# Autodesk Inventor assembly: Anemometr
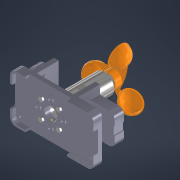
[picture p0: Inventor's stored thumbnail of the model, 180x180]
Saved by Autodesk Inventor 2021.2 (Build 252289000, 289)
## iProperties
Created: 2021-10-17
Part Number: Anemometr
Document SubType Name: Assembly
Designer: DuctopwH
Author: DuctopwH
## Documents named in this file (18)
- F:\Projects\cadblueprints\002-АНМ\002-ANM.iam
- F:\Projects\cadblueprints\002-АНМ\parts\002.10-plita.ipt
- F:\Projects\cadblueprints\002-АНМ\parts\002.09-flanec.ipt
- F:\Projects\cadblueprints\002-АНМ\parts\002.01-korpus.ipt
- F:\Projects\cadblueprints\002-АНМ\parts\002.02-osnovanie.ipt
- C:\Users\DuctopwH\Documents\Inventor\Content Center Files\R2021\en-US\Bolt GOST R 50274-92\Bolt M5-6g×16-F GOST R 50274-92.ipt
- F:\Projects\cadblueprints\002-АНМ\parts\002.04-terminal.ipt
- C:\Users\DuctopwH\Documents\Inventor\Content Center Files\R2021\en-US\GOST 10450-78\Washer 2,7 GOST 10450-78.ipt
- C:\Users\DuctopwH\Documents\Inventor\Content Center Files\R2021\en-US\GOST 5916-70\Nut M2,5-6H GOST 5916-70.ipt
- F:\Projects\cadblueprints\002-АНМ\parts\002.08-kryshka.ipt
- F:\Projects\cadblueprints\002-АНМ\standard-parts\ANSI B18.3.1M - M2,5x0,45 x 12.ipt
- F:\Projects\cadblueprints\002-АНМ\standard-parts\DIN 988 - S4 x 8.ipt
- F:\Projects\cadblueprints\002-АНМ\parts\002.06-rotor.ipt
- F:\Projects\cadblueprints\002-АНМ\parts\002.05-val.ipt
- F:\Projects\cadblueprints\002-АНМ\parts\002.03-vtulka.ipt
- F:\Projects\cadblueprints\002-АНМ\standard-parts\Ring 8 GOST 13943-86.ipt
- F:\Projects\cadblueprints\002-АНМ\parts\002.07-krylchatka.ipt
- C:\Users\DuctopwH\Documents\Inventor\Content Center Files\R2021\en-US\Bolt GOST R 50792-95\Bolt M5×20 GOST R 50792-95.ipt
## Components (26 placed, 17 different names)
1. 002.10-plita:1 — Mate:1, Flush:1, Flush:2, Mate:2, Mate:3, Mate:4, Mate:6, Mate:7, Insert:3, Insert:4, Insert:5, Insert:6
2. 002.09-flanec:1 — Mate:2, Mate:3, Mate:4, Mate:5
3. 002.01-korpus:1 — Mate:5, Mate:6, Mate:7, Mate:8, Mate:9, Mate:10, Insert:1, Insert:2, Mate:25, Mate:26, Mate:27, Mate:29, Mate:31
4. 002.02-osnovanie:1 — Mate:8, Mate:9, Mate:10, Mate:11, Mate:12, Mate:15, Mate:16, Mate:18, Mate:20, Mate:32, Mate:33, Mate:34, Mate:38, Mate:49, Mate:50
5. Bolt GOST R 50274-92 M5-6g×16-F:1 — Insert:1
6. Bolt GOST R 50274-92 M5-6g×16-F:2 — Insert:2
7. 002.04-terminal:1 — Mate:12, Mate:16, Mate:19, Mate:23, Mate:49
8. 002.04-terminal:2 — Mate:11, Mate:15, Mate:17, Mate:21, Mate:50
9. Washer GOST 10450-78 2,7:1 — Mate:17, Mate:18, Mate:22
10. Washer GOST 10450-78 2,7:2 — Mate:19, Mate:20, Mate:24
11. Nut GOST 5916-70 M2,5:1 — Mate:21, Mate:22
12. Nut GOST 5916-70 M2,5:2 — Mate:23, Mate:24
13. 002.08-kryshka:1 — Mate:25, Mate:26, Mate:27, Mate:28, Mate:30, Flush:3, Mate:42, Mate:43, Mate:46, Mate:48
14. Broached Socket Head Cap Screw - Metric M2,5x0,45 x 12:1 — Mate:28, Mate:29
15. Broached Socket Head Cap Screw - Metric M2,5x0,45 x 12:2 — Mate:30, Mate:31
16. DIN 988 S4 x 8:1 — Mate:32, Mate:33, Mate:36
17. 002.06-rotor:1 — Mate:34, Mate:35, Mate:36
18. 002.05-val:1 — Mate:38, Mate:39, Mate:40, Mate:44
19. 002.03-vtulka:1 — Mate:39, Flush:3, Mate:41
20. 002.03-vtulka:2 — Mate:40, Mate:41
21. Ring GOST 13943-86 A 8:1 — Mate:47, Mate:48
22. 002.07-krylchatka:1 — Mate:42, Mate:43, Mate:44, Mate:46, Mate:47
23. Bolt GOST R 50792-95 M5×20:1 — Insert:3
24. Bolt GOST R 50792-95 M5×20:2 — Insert:4
25. Bolt GOST R 50792-95 M5×20:3 — Insert:5
26. Bolt GOST R 50792-95 M5×20:4 — Insert:6
## Relationships (55: Mate 46, Insert 6, Flush 3)
- Mate:1: 002.10-plita:1
- Flush:1: 002.10-plita:1
- Flush:2: 002.10-plita:1
- Mate:2: 002.10-plita:1 ↔ 002.09-flanec:1
- Mate:3: 002.10-plita:1 ↔ 002.09-flanec:1
- Mate:4: 002.10-plita:1 ↔ 002.09-flanec:1
- Mate:5: 002.09-flanec:1 ↔ 002.01-korpus:1
- Mate:6: 002.10-plita:1 ↔ 002.01-korpus:1
- Mate:7: 002.10-plita:1 ↔ 002.01-korpus:1
- Mate:8: 002.01-korpus:1 ↔ 002.02-osnovanie:1
- Mate:9: 002.01-korpus:1 ↔ 002.02-osnovanie:1
- Mate:10: 002.01-korpus:1 ↔ 002.02-osnovanie:1
- Insert:1: 002.01-korpus:1 ↔ Bolt GOST R 50274-92 M5-6g×16-F:1
- Insert:2: 002.01-korpus:1 ↔ Bolt GOST R 50274-92 M5-6g×16-F:2
- Mate:11: 002.02-osnovanie:1 ↔ 002.04-terminal:2
- Mate:12: 002.02-osnovanie:1 ↔ 002.04-terminal:1
- Mate:15: 002.02-osnovanie:1 ↔ 002.04-terminal:2
- Mate:16: 002.02-osnovanie:1 ↔ 002.04-terminal:1
- Mate:17: 002.04-terminal:2 ↔ Washer GOST 10450-78 2,7:1
- Mate:18: 002.02-osnovanie:1 ↔ Washer GOST 10450-78 2,7:1
- Mate:19: 002.04-terminal:1 ↔ Washer GOST 10450-78 2,7:2
- Mate:20: 002.02-osnovanie:1 ↔ Washer GOST 10450-78 2,7:2
- Mate:21: 002.04-terminal:2 ↔ Nut GOST 5916-70 M2,5:1
- Mate:22: Washer GOST 10450-78 2,7:1 ↔ Nut GOST 5916-70 M2,5:1
- Mate:23: 002.04-terminal:1 ↔ Nut GOST 5916-70 M2,5:2
- Mate:24: Washer GOST 10450-78 2,7:2 ↔ Nut GOST 5916-70 M2,5:2
- Mate:25: 002.01-korpus:1 ↔ 002.08-kryshka:1
- Mate:26: 002.01-korpus:1 ↔ 002.08-kryshka:1
- Mate:27: 002.01-korpus:1 ↔ 002.08-kryshka:1
- Mate:28: 002.08-kryshka:1 ↔ Broached Socket Head Cap Screw - Metric M2,5x0,45 x 12:1
- Mate:29: 002.01-korpus:1 ↔ Broached Socket Head Cap Screw - Metric M2,5x0,45 x 12:1
- Mate:30: 002.08-kryshka:1 ↔ Broached Socket Head Cap Screw - Metric M2,5x0,45 x 12:2
- Mate:31: 002.01-korpus:1 ↔ Broached Socket Head Cap Screw - Metric M2,5x0,45 x 12:2
- Mate:32: 002.02-osnovanie:1 ↔ DIN 988 S4 x 8:1
- Mate:33: 002.02-osnovanie:1 ↔ DIN 988 S4 x 8:1
- Mate:34: 002.02-osnovanie:1 ↔ 002.06-rotor:1
- Mate:35: 002.06-rotor:1
- Mate:36: DIN 988 S4 x 8:1 ↔ 002.06-rotor:1
- Mate:38: 002.02-osnovanie:1 ↔ 002.05-val:1
- Mate:39: 002.05-val:1 ↔ 002.03-vtulka:1
- Mate:40: 002.05-val:1 ↔ 002.03-vtulka:2
- Flush:3: 002.08-kryshka:1 ↔ 002.03-vtulka:1
- Mate:41: 002.03-vtulka:1 ↔ 002.03-vtulka:2
- Mate:42: 002.08-kryshka:1 ↔ 002.07-krylchatka:1
- Mate:43: 002.08-kryshka:1 ↔ 002.07-krylchatka:1
- Mate:44: 002.05-val:1 ↔ 002.07-krylchatka:1
- Mate:46: 002.08-kryshka:1 ↔ 002.07-krylchatka:1
- Mate:47: Ring GOST 13943-86 A 8:1 ↔ 002.07-krylchatka:1
- Mate:48: 002.08-kryshka:1 ↔ Ring GOST 13943-86 A 8:1
- Mate:49: 002.02-osnovanie:1 ↔ 002.04-terminal:1
- Mate:50: 002.02-osnovanie:1 ↔ 002.04-terminal:2
- Insert:3: 002.10-plita:1 ↔ Bolt GOST R 50792-95 M5×20:1
- Insert:4: 002.10-plita:1 ↔ Bolt GOST R 50792-95 M5×20:2
- Insert:5: 002.10-plita:1 ↔ Bolt GOST R 50792-95 M5×20:3
- Insert:6: 002.10-plita:1 ↔ Bolt GOST R 50792-95 M5×20:4
